# Autodesk Inventor assembly: Steering Assembly
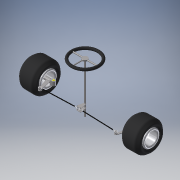
[picture p0: Inventor's stored thumbnail of the model, 180x180]
Saved by Autodesk Inventor 2016 (Build 200138000, 138)
## iProperties
Created: 2015-06-02
Part Number: Steering Assembly
Document SubType Name: Assembly
Designer: Dennis
Author: Dennis
## Documents named in this file (11)
- C:\Users\Matthew Cheung\Dropbox\Work\National Instruments\Shared Folder\Steering\Steering Assembly.iam
- C:\Users\Matthew Cheung\Dropbox\Work\National Instruments\Shared Folder\Steering\Steering Wheel and Rod.ipt
- C:\Users\Matthew Cheung\Dropbox\Work\National Instruments\Shared Folder\Steering\Tie Rod to Front Axle Connecting Plate.ipt
- C:\Users\Matthew Cheung\Dropbox\Work\National Instruments\Shared Folder\Steering\Tie Rod.ipt
- C:\Users\Matthew Cheung\Dropbox\Work\National Instruments\Shared Folder\Steering\Tie Rod to Front Axle Connecting Plate_MIR.ipt
- C:\Users\Matthew Cheung\Dropbox\Work\National Instruments\Shared Folder\Steering\Tie Rod_MIR.ipt
- C:\Users\Matthew Cheung\Dropbox\Work\National Instruments\Shared Folder\Steering\Wheel Hub.ipt
- C:\Users\Matthew Cheung\Dropbox\Work\National Instruments\Shared Folder\Steering\Wheel Tire.ipt
- C:\Users\Matthew Cheung\Dropbox\Work\National Instruments\Shared Folder\Steering\Wheel Hub_MIR.ipt
- C:\Users\Matthew Cheung\Dropbox\Work\National Instruments\Shared Folder\Steering\Wheel Tire_MIR.ipt
- C:\Users\Matthew Cheung\Dropbox\Work\National Instruments\Shared Folder\Steering\Motor Black Box.ipt
## Components (10 placed, 10 different names)
1. Steering Wheel and Rod:1 — Mate:1, Mate:7, Mate:13, Mate:19, Flush:4, Flush:5, Mate:33, Mate:34
2. Wheel Hub_MIR:1 — Mate:29, Mate:30, Mate:32, Flush:6
3. Wheel Tire_MIR:1 — Mate:29, Mate:30
4. Motor Black Box:1 — Mate:33, Angle:3, Mate:34
5. Tie Rod to Front Axle Connecting Plate:1 — Mate:4, Angle:1, Flush:16, Mate:8, Mate:9, Mate:12, Mate:27, Flush:7
6. Tie Rod:1 — Mate:4, Flush:16, Mate:13, Flush:4
7. Tie Rod to Front Axle Connecting Plate_MIR:1 — Angle:2, Flush:15, Mate:15, Mate:16, Mate:17, Mate:23, Mate:32, Flush:6
8. Tie Rod_MIR:1 — Flush:15, Mate:15, Mate:19, Flush:5
9. Wheel Hub:1 — Mate:25, Mate:26, Mate:27, Flush:7
10. Wheel Tire:1 — Mate:25, Mate:26
## Relationships (36: Mate 24, Flush 9, Angle 3)
- Mate:1: Steering Wheel and Rod:1
- Mate:4: Tie Rod to Front Axle Connecting Plate:1 ↔ Tie Rod:1
- Angle:1 (0 deg): Tie Rod to Front Axle Connecting Plate:1
- Flush:16: Tie Rod to Front Axle Connecting Plate:1 ↔ Tie Rod:1
- Mate:7: Steering Wheel and Rod:1
- Mate:8: Tie Rod to Front Axle Connecting Plate:1
- Mate:9: Tie Rod to Front Axle Connecting Plate:1
- Flush:1 (361.95 mm)
- Flush:2 (-57.15 mm)
- Mate:10
- Mate:11
- Mate:12: Tie Rod to Front Axle Connecting Plate:1
- Mate:13: Steering Wheel and Rod:1 ↔ Tie Rod:1
- Angle:2 (0 deg): Tie Rod to Front Axle Connecting Plate_MIR:1
- Flush:15: Tie Rod to Front Axle Connecting Plate_MIR:1 ↔ Tie Rod_MIR:1
- Mate:15: Tie Rod to Front Axle Connecting Plate_MIR:1 ↔ Tie Rod_MIR:1
- Mate:16: Tie Rod to Front Axle Connecting Plate_MIR:1
- Mate:17: Tie Rod to Front Axle Connecting Plate_MIR:1
- Mate:19: Steering Wheel and Rod:1 ↔ Tie Rod_MIR:1
- Flush:3 (-361.95 mm)
- Mate:21
- Mate:22
- Mate:23: Tie Rod to Front Axle Connecting Plate_MIR:1
- Mate:25: Wheel Hub:1 ↔ Wheel Tire:1
- Mate:26: Wheel Hub:1 ↔ Wheel Tire:1
- Mate:27: Tie Rod to Front Axle Connecting Plate:1 ↔ Wheel Hub:1
- Mate:29: Wheel Hub_MIR:1 ↔ Wheel Tire_MIR:1
- Mate:30: Wheel Hub_MIR:1 ↔ Wheel Tire_MIR:1
- Flush:4: Steering Wheel and Rod:1 ↔ Tie Rod:1
- Flush:5: Steering Wheel and Rod:1 ↔ Tie Rod_MIR:1
- Mate:32: Wheel Hub_MIR:1 ↔ Tie Rod to Front Axle Connecting Plate_MIR:1
- Flush:6: Wheel Hub_MIR:1 ↔ Tie Rod to Front Axle Connecting Plate_MIR:1
- Flush:7: Tie Rod to Front Axle Connecting Plate:1 ↔ Wheel Hub:1
- Mate:33: Steering Wheel and Rod:1 ↔ Motor Black Box:1
- Angle:3 (0 deg): Motor Black Box:1
- Mate:34 (50.8 mm): Steering Wheel and Rod:1 ↔ Motor Black Box:1
